# Autodesk Inventor assembly: sPhenixTileTestStand-Tile9
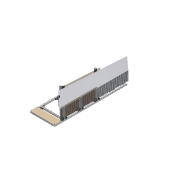
[picture p0: Inventor's stored thumbnail of the model, 180x180]
Saved by Autodesk Inventor 2018 (Build 220112000, 112)
## iProperties
Created: 2017-03-01
Part Number: sPhenixTileTestStand-Tile9
Document SubType Name: Assembly
Designer: sawaiz
Author: sawaiz
## Documents named in this file (16)
- C:\Users\sawaiz\OneDrive\projects\sPhenixTileTestStand\sPhenixTileTestStand.iam
- C:\Users\sawaiz\oneDrive\projects\sPhenixTileTestStand\frame\staticFrame.iam
- C:\Users\sawaiz\oneDrive\projects\sPhenixTileTestStand\tiles\outerHCAL\OuterHCALtile9.ipt
- C:\Users\sawaiz\oneDrive\projects\sPhenixTileTestStand\tiles\outerHCAL.ipt
- C:\Users\sawaiz\oneDrive\projects\sPhenixTileTestStand\frame\hfs5-2020Height.ipt
- C:\Users\sawaiz\oneDrive\projects\sPhenixTileTestStand\hardware\angleBracket.iam
- C:\Users\sawaiz\oneDrive\projects\sPhenixTileTestStand\hardware\HHPFLN5-1.ipt
- C:\Users\sawaiz\oneDrive\projects\sPhenixTileTestStand\hardware\HHPFRN5-1.ipt
- C:\Users\sawaiz\oneDrive\projects\sPhenixTileTestStand\hardware\HHPFRN5-2.ipt
- C:\Users\sawaiz\oneDrive\projects\sPhenixTileTestStand\hardware\HHPFLN5-2.ipt
- C:\Users\sawaiz\oneDrive\projects\sPhenixTileTestStand\frame\wallPlate.ipt
- sPhenixTileTestStand-Tile10.iam
- sPhenixTileTestStand-Tile11.iam
- sPhenixTileTestStand-Tile12.iam
- sPhenixTileTestStand-Tile9.iam
- C:\Users\sawaiz\oneDrive\projects\sPhenixTileTestStand\sPhenixTileTestStand.xlsx
## Components (26 placed, 9 different names)
1. staticFrame:1 [sub-assembly] — Flush:5, Flush:6, Mate:5, Mate:13, Mate:14
2. hfs5-2020Height:1 — Mate:3, Flush:1, Flush:2, Flush:7, Mate:7, Angle:1, Mate:9, Flush:12, Flush:14, Mate:15
3. hfs5-2020Height:2 — Mate:4, Flush:3, Flush:4, Flush:7, Mate:6, Mate:8
4. angleBracket:1 [sub-assembly] — Mate:3, Flush:1, Flush:2, Flush:6, Mate:5
5. angleBracket:2 [sub-assembly] — Mate:4, Flush:3, Flush:4, Flush:5
6. HHPFLN5-1:1 — Mate:7, Angle:1, Angle:2, Mate:9, Flush:9, Mate:11, Flush:11, Flush:12
7. HHPFRN5-1:1 — Mate:6, Angle:2, Mate:8, Flush:9, Mate:10, Flush:10
8. HHPFRN5-2:1 — Mate:10, Flush:10, Flush:13, Mate:12
9. HHPFLN5-2:1 — Mate:11, Flush:11, Flush:13
10. wallPlate:1 — Mate:12, Flush:14, Mate:15, Mate:16
11. OuterHCALtile9:1 — Mate:13, Mate:14, Mate:16
12. OuterHCALtile9:2
13. OuterHCALtile9:3
14. OuterHCALtile9:4
15. OuterHCALtile9:5
16. OuterHCALtile9:6
17. OuterHCALtile9:7
18. OuterHCALtile9:8
19. OuterHCALtile9:9
20. OuterHCALtile9:10
21. OuterHCALtile9:11
22. OuterHCALtile9:12
23. OuterHCALtile9:13
24. OuterHCALtile9:14
25. OuterHCALtile9:15
26. OuterHCALtile9:16
## Component patterns: (16 elements, first: OuterHCALtile9:1)
## Relationships (29: Mate 14, Flush 13, Angle 2)
- Mate:3: hfs5-2020Height:1 ↔ angleBracket:1
- Flush:1: hfs5-2020Height:1 ↔ angleBracket:1
- Flush:2: hfs5-2020Height:1 ↔ angleBracket:1
- Mate:4: hfs5-2020Height:2 ↔ angleBracket:2
- Flush:3: hfs5-2020Height:2 ↔ angleBracket:2
- Flush:4: hfs5-2020Height:2 ↔ angleBracket:2
- Flush:5: staticFrame:1 ↔ angleBracket:2
- Flush:6: staticFrame:1 ↔ angleBracket:1
- Flush:7: hfs5-2020Height:1 ↔ hfs5-2020Height:2
- Mate:5: staticFrame:1 ↔ angleBracket:1
- Mate:6: hfs5-2020Height:2 ↔ HHPFRN5-1:1
- Mate:7: hfs5-2020Height:1 ↔ HHPFLN5-1:1
- Angle:1 (0 deg): hfs5-2020Height:1 ↔ HHPFLN5-1:1
- Angle:2 (0 deg): HHPFLN5-1:1 ↔ HHPFRN5-1:1
- Mate:8 (3 mm): hfs5-2020Height:2 ↔ HHPFRN5-1:1
- Mate:9 (3 mm): hfs5-2020Height:1 ↔ HHPFLN5-1:1
- Flush:9: HHPFLN5-1:1 ↔ HHPFRN5-1:1
- Mate:10: HHPFRN5-1:1 ↔ HHPFRN5-2:1
- Flush:10: HHPFRN5-1:1 ↔ HHPFRN5-2:1
- Mate:11: HHPFLN5-1:1 ↔ HHPFLN5-2:1
- Flush:11: HHPFLN5-1:1 ↔ HHPFLN5-2:1
- Flush:12: hfs5-2020Height:1 ↔ HHPFLN5-1:1
- Flush:13: HHPFRN5-2:1 ↔ HHPFLN5-2:1
- Mate:12: HHPFRN5-2:1 ↔ wallPlate:1
- Flush:14: hfs5-2020Height:1 ↔ wallPlate:1
- Mate:13: staticFrame:1 ↔ OuterHCALtile9:1
- Mate:14: staticFrame:1 ↔ OuterHCALtile9:1
- Mate:15: hfs5-2020Height:1 ↔ wallPlate:1
- Mate:16: wallPlate:1 ↔ OuterHCALtile9:1
## Named parameters: width = 300 mm, depth = 1000 mm, height = 150 mm, suppourtPlateLength = 100 mm, acrylicThickness = 3.125 mm
